# Autodesk Inventor assembly: mill_assembly
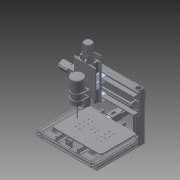
[picture p0: Inventor's stored thumbnail of the model, 180x180]
Saved by Autodesk Inventor 2014 (Build 180170000, 170)
## iProperties
Created: 2014-08-08
Part Number: mill_assembly
Document SubType Name: Assembly
Designer: Matthew
Author: Matthew
## Documents named in this file (29)
- C:\Users\Matthew\Documents\GitHub\CNC Mill\mill_assembly.iam
- C:\Users\Matthew\Documents\GitHub\CNC Mill\Imported Components\8020-2040\Assembly2.iam
- C:\Users\Matthew\Documents\GitHub\CNC Mill\8020\2020.ipt
- C:\Users\Matthew\Documents\GitHub\CNC Mill\8020\2020_18in.ipt
- C:\Users\Matthew\Documents\GitHub\CNC Mill\plate_4127.ipt
- C:\Users\Matthew\Documents\GitHub\CNC Mill\8020\gusset_4138.ipt
- C:\Users\Matthew\Documents\GitHub\CNC Mill\8020\gusset_4134.ipt
- C:\Users\Matthew\Documents\GitHub\CNC Mill\mic6_plate.ipt
- C:\Users\Matthew\Documents\GitHub\CNC Mill\1605\1605_400mm.ipt
- C:\Users\Matthew\Documents\GitHub\CNC Mill\1605\1605_ballnut.ipt
- C:\Users\Matthew\Documents\GitHub\CNC Mill\nema23_motor_mount.ipt
- C:\Users\Matthew\Documents\GitHub\CNC Mill\fk12.ipt
- C:\Users\Matthew\Documents\GitHub\CNC Mill\sbr\sbr20\SBR20UU.iam
- C:\Users\Matthew\Documents\GitHub\CNC Mill\6.35x10mm_coupler.ipt
- C:\Users\Matthew\Documents\GitHub\CNC Mill\sbr\sbr20\sbr20_400mm.ipt
- C:\Users\Matthew\Documents\GitHub\CNC Mill\HD16.ipt
- C:\Users\Matthew\Documents\GitHub\CNC Mill\nema23_HS8630.ipt
- C:\Users\Matthew\Documents\GitHub\CNC Mill\z-axis_mount_plate.ipt
- C:\Users\Matthew\Documents\GitHub\CNC Mill\1605\1605_200mm.ipt
- C:\Users\Matthew\Documents\GitHub\CNC Mill\y-axis_mount_plate.ipt
- C:\Users\Matthew\Documents\GitHub\CNC Mill\8020\2020_16in.ipt
- C:\Users\Matthew\Documents\GitHub\CNC Mill\router_plate.ipt
- C:\Users\Matthew\Documents\GitHub\CNC Mill\router_mount.ipt
- C:\Users\Matthew\Documents\GitHub\CNC Mill\1617evs.ipt
- C:\Users\Matthew\Documents\GitHub\CNC Mill\ff12_mount.ipt
- C:\Users\Matthew\Documents\GitHub\CNC Mill\ff12.ipt
- C:\Users\Matthew\Documents\GitHub\CNC Mill\sbr\sbr20\sbr20_500mm.ipt
- C:\Users\Matthew\Documents\GitHub\CNC Mill\1605\1605_500mm.ipt
- C:\Users\Matthew\Documents\GitHub\CNC Mill\sbr\sbr20\sbr20_300mm.ipt
## Components (69 placed, 28 different names)
1. Assembly2:1 [sub-assembly] — Mate:22, Mate:24, Mate:26, Mate:39, Mate:41, Mate:42, Mate:43, Mate:45, Mate:161, Flush:91, Flush:114, Flush:115, Mate:184, Flush:117, Flush:118
2. 2020_18in:1 — Mate:31, Mate:32, Mate:38, Mate:47, Mate:48, Mate:181, Flush:107, Flush:113, Flush:127, Mate:192, Flush:128
3. 2020_18in:2 — Mate:28, Mate:29, Mate:34, Mate:50, Mate:51, Mate:189, Flush:124, Flush:125
4. plate_4127:1 — Mate:39, Mate:41, Flush:119
5. gusset_4138:1 — Mate:22
6. gusset_4134:1 — Mate:28, Mate:29
7. gusset_4138:2 — Mate:24, Mate:26, Mate:207
8. gusset_4134:2 — Mate:31, Mate:32
9. gusset_4134:3 — Mate:34, Flush:61, Mate:193
10. gusset_4134:4 — Mate:38, Flush:62, Mate:191
11. plate_4127:2 — Mate:42, Mate:43, Mate:45, Flush:116
12. gusset_4134:5 — Mate:50, Mate:51
13. gusset_4134:6 — Mate:47, Mate:48, Flush:61, Flush:62
14. mic6_plate:1 — Flush:76, Flush:77, Mate:141
15. 1605_400mm:1 — Mate:98, Mate:100, Mate:108, Insert:2, Insert:13
16. 1605_ballnut:1 — Mate:108, Mate:133, Mate:134, Flush:75
17. nema23_motor_mount:1 — Mate:99, Mate:136, Mate:137, Mate:196, Flush:132
18. nema23_motor_mount:2 — Mate:153, Flush:86, Mate:154, Mate:155, Mate:156, Mate:157
19. 1605_ballnut:6 — Mate:150, Mate:158, Flush:90, Mate:159
20. fk12:1 — Mate:98, Mate:99, Mate:100, Mate:137
21. fk12:3 — Mate:156, Mate:157, Mate:214
22. SBR20UU:1 [sub-assembly] — Mate:131, Flush:69, Flush:70, Flush:73, Mate:138, Mate:140, Flush:77, Mate:141
23. 6.35x10mm_coupler:1 — Insert:3, Insert:4
24. sbr20_400mm:1 — Mate:130, Mate:198, Flush:136
25. SBR20UU:2 [sub-assembly] — Mate:129, Mate:132, Flush:71, Flush:72, Mate:139
26. sbr20_400mm:2 — Mate:129, Mate:197, Flush:136
27. SBR20UU:3 [sub-assembly] — Mate:130, Mate:131, Flush:69, Flush:70, Flush:74, Flush:76
28. SBR20UU:4 [sub-assembly] — Mate:132, Flush:71, Flush:72, Flush:73, Flush:74
29. HD16:1 — Mate:133, Mate:134, Flush:75, Mate:138, Mate:139, Mate:140
30. nema23_HS8630:1 — Mate:135, Mate:136
31. 6.35x10mm_coupler:2 — Insert:2, Mate:135
32. SBR20UU:5 [sub-assembly] — Flush:78, Flush:79, Mate:144, Flush:84, Flush:85, Mate:160
33. SBR20UU:6 [sub-assembly] — Flush:78, Flush:79, Mate:144, Mate:213
34. SBR20UU:7 [sub-assembly] — Flush:84, Flush:85
35. SBR20UU:8 [sub-assembly] — Mate:212
36. z-axis_mount_plate:1 — Mate:153, Flush:86, Mate:167, Flush:102, Flush:103, Mate:208, Mate:209, Flush:139
37. 1605_200mm:1 — Mate:150, Insert:3
38. nema23_HS8630:2 — Mate:154, Mate:155, Insert:4
39. HD16:6 — Mate:158, Flush:90, Mate:159, Mate:160, Mate:186, Flush:120, Flush:121, Mate:210, Mate:211
40. y-axis_mount_plate:1 — Mate:161, Flush:91, Mate:177, Mate:199, Mate:200, Flush:135, Mate:206, Flush:137
41. SBR20UU:9 [sub-assembly] — Flush:95, Flush:96, Flush:99, Flush:101, Mate:167, Flush:103, Mate:201
42. SBR20UU:10 [sub-assembly] — Flush:95, Flush:96, Mate:166, Flush:97, Flush:98, Flush:102
43. SBR20UU:11 [sub-assembly] — Flush:99, Flush:100, Flush:101
44. SBR20UU:12 [sub-assembly] — Mate:166, Flush:97, Flush:98, Flush:100, Mate:180, Mate:202
45. nema23_motor_mount:4 — Mate:177, Flush:137
46. fk12:4 — Insert:8, Mate:204, Insert:10
47. 6.35x10mm_coupler:3
48. nema23_HS8630:3
49. 1605_400mm:2 — Mate:176, Insert:8
50. 1605_ballnut:7 — Mate:176
51. HD16:7 — Mate:180, Mate:203, Mate:205
52. 2020_16in:1 — Mate:181, Flush:107, Flush:113, Flush:114, Flush:115, Mate:184, Flush:116, Mate:194, Flush:129, Flush:130, Mate:207
53. 2020_16in:2 — Flush:117, Flush:118, Flush:119, Mate:195, Flush:131
54. router_plate:1 — Mate:186, Flush:120, Flush:121, Mate:187, Flush:122, Flush:123
55. router_mount:1 — Insert:7, Mate:187, Flush:122, Flush:123
56. 1617evs:1 — Insert:7
57. ff12_mount:1 — Insert:9
58. ff12:1 — Insert:9, Insert:13
59. sbr20_500mm:1 — Flush:133, Mate:200, Mate:201, Mate:203, Mate:204, Flush:135
60. 2020_16in:3 — Mate:189, Flush:124, Flush:125, Flush:127, Mate:191, Mate:192, Flush:128, Mate:193, Mate:197, Mate:198, Mate:215, Mate:216, Flush:141
61. 2020_16in:4 — Mate:194, Flush:129, Flush:130, Mate:195, Flush:131, Mate:196, Flush:132, Flush:140
62. sbr20_500mm:2 — Flush:133, Mate:199, Mate:202, Mate:205
63. 1605_500mm:1 — Insert:10, Insert:11
64. ff12:2 — Insert:11, Insert:12
65. ff12_mount:2 — Insert:12, Mate:206
66. sbr20_300mm:1 — Flush:138, Mate:208, Mate:210, Mate:213, Mate:214, Flush:139
67. sbr20_300mm:2 — Flush:138, Mate:209, Mate:211, Mate:212
68. 2020:1 — Mate:215, Flush:140
69. 2020:2 — Mate:216, Flush:141
## Relationships (158: Mate 89, Flush 58, Insert 11)
- Mate:22: Assembly2:1 ↔ gusset_4138:1
- Mate:24: Assembly2:1 ↔ gusset_4138:2
- Mate:26: Assembly2:1 ↔ gusset_4138:2
- Mate:28: 2020_18in:2 ↔ gusset_4134:1
- Mate:29: 2020_18in:2 ↔ gusset_4134:1
- Mate:31: 2020_18in:1 ↔ gusset_4134:2
- Mate:32: 2020_18in:1 ↔ gusset_4134:2
- Mate:34: 2020_18in:2 ↔ gusset_4134:3
- Mate:38: 2020_18in:1 ↔ gusset_4134:4
- Mate:39: Assembly2:1 ↔ plate_4127:1
- Mate:41: Assembly2:1 ↔ plate_4127:1
- Mate:42: Assembly2:1 ↔ plate_4127:2
- Mate:43: Assembly2:1 ↔ plate_4127:2
- Mate:45: Assembly2:1 ↔ plate_4127:2
- Mate:47: 2020_18in:1 ↔ gusset_4134:6
- Mate:48: 2020_18in:1 ↔ gusset_4134:6
- Mate:50: 2020_18in:2 ↔ gusset_4134:5
- Mate:51: 2020_18in:2 ↔ gusset_4134:5
- Mate:98: 1605_400mm:1 ↔ fk12:1
- Mate:99: nema23_motor_mount:1 ↔ fk12:1
- Mate:100: 1605_400mm:1 ↔ fk12:1
- Mate:108: 1605_400mm:1 ↔ 1605_ballnut:1
- Flush:61: gusset_4134:3 ↔ gusset_4134:6
- Flush:62: gusset_4134:4 ↔ gusset_4134:6
- Mate:129: SBR20UU:2 ↔ sbr20_400mm:2
- Mate:130: sbr20_400mm:1 ↔ SBR20UU:3
- Mate:131 (20 mm): SBR20UU:1 ↔ SBR20UU:3
- Flush:69: SBR20UU:1 ↔ SBR20UU:3
- Flush:70: SBR20UU:1 ↔ SBR20UU:3
- Mate:132 (20 mm): SBR20UU:2 ↔ SBR20UU:4
- Flush:71: SBR20UU:2 ↔ SBR20UU:4
- Flush:72: SBR20UU:2 ↔ SBR20UU:4
- Flush:73: SBR20UU:1 ↔ SBR20UU:4
- Flush:74: SBR20UU:3 ↔ SBR20UU:4
- Mate:133: 1605_ballnut:1 ↔ HD16:1
- Mate:134: 1605_ballnut:1 ↔ HD16:1
- Flush:75: 1605_ballnut:1 ↔ HD16:1
- Insert:2 (-12.5 mm): 1605_400mm:1 ↔ 6.35x10mm_coupler:2
- Mate:135: nema23_HS8630:1 ↔ 6.35x10mm_coupler:2
- Mate:136: nema23_motor_mount:1 ↔ nema23_HS8630:1
- Mate:137: nema23_motor_mount:1 ↔ fk12:1
- Mate:138 (42.3 mm): SBR20UU:1 ↔ HD16:1
- Mate:139 (42.3 mm): SBR20UU:2 ↔ HD16:1
- Mate:140 (-7.5 mm): SBR20UU:1 ↔ HD16:1
- Flush:76 (38.1 mm): mic6_plate:1 ↔ SBR20UU:3
- Flush:77 (-92.4052 mm): mic6_plate:1 ↔ SBR20UU:1
- Mate:141: mic6_plate:1 ↔ SBR20UU:1
- Flush:78: SBR20UU:5 ↔ SBR20UU:6
- Flush:79: SBR20UU:5 ↔ SBR20UU:6
- Mate:144 (10 mm): SBR20UU:5 ↔ SBR20UU:6
- [Flush]: SBR20UU:7 ↔ SBR20UU:8
- [Flush]: SBR20UU:7 ↔ SBR20UU:8
- [Mate] (10 mm): SBR20UU:7 ↔ SBR20UU:8
- Flush:84: SBR20UU:5 ↔ SBR20UU:7
- Flush:85: SBR20UU:5 ↔ SBR20UU:7
- Mate:150: 1605_ballnut:6 ↔ 1605_200mm:1
- Insert:3 (-12.5 mm): 6.35x10mm_coupler:1 ↔ 1605_200mm:1
- Mate:153: nema23_motor_mount:2 ↔ z-axis_mount_plate:1
- Flush:86: nema23_motor_mount:2 ↔ z-axis_mount_plate:1
- Mate:154: nema23_motor_mount:2 ↔ nema23_HS8630:2
- Mate:155: nema23_motor_mount:2 ↔ nema23_HS8630:2
- Insert:4 (-7 mm): 6.35x10mm_coupler:1 ↔ nema23_HS8630:2
- Mate:156: nema23_motor_mount:2 ↔ fk12:3
- Mate:157: nema23_motor_mount:2 ↔ fk12:3
- Mate:158: 1605_ballnut:6 ↔ HD16:6
- Flush:90: 1605_ballnut:6 ↔ HD16:6
- Mate:159: 1605_ballnut:6 ↔ HD16:6
- Mate:160 (-12.5 mm): SBR20UU:5 ↔ HD16:6
- Mate:161: Assembly2:1 ↔ y-axis_mount_plate:1
- Flush:91: Assembly2:1 ↔ y-axis_mount_plate:1
- Flush:95: SBR20UU:9 ↔ SBR20UU:10
- Flush:96: SBR20UU:9 ↔ SBR20UU:10
- Mate:166 (60 mm): SBR20UU:10 ↔ SBR20UU:12
- Flush:97: SBR20UU:10 ↔ SBR20UU:12
- Flush:98: SBR20UU:10 ↔ SBR20UU:12
- Flush:99: SBR20UU:9 ↔ SBR20UU:11
- Flush:100: SBR20UU:11 ↔ SBR20UU:12
- Flush:101: SBR20UU:9 ↔ SBR20UU:11
- Mate:167: z-axis_mount_plate:1 ↔ SBR20UU:9
- Flush:102: z-axis_mount_plate:1 ↔ SBR20UU:10
- Flush:103: z-axis_mount_plate:1 ↔ SBR20UU:9
- [Mate]: nema23_motor_mount:4 ↔ nema23_HS8630:3
- [Mate]: nema23_motor_mount:4 ↔ nema23_HS8630:3
- [Insert] (-7 mm): 6.35x10mm_coupler:3 ↔ nema23_HS8630:3
- [Mate]: nema23_motor_mount:4 ↔ fk12:4
- [Mate]: nema23_motor_mount:4 ↔ fk12:4
- [Mate]: 1605_ballnut:7 ↔ HD16:7
- [Flush]: 1605_ballnut:7 ↔ HD16:7
- [Mate]: 1605_ballnut:7 ↔ HD16:7
- Mate:176: 1605_400mm:2 ↔ 1605_ballnut:7
- Mate:177: y-axis_mount_plate:1 ↔ nema23_motor_mount:4
- Mate:180 (12.5 mm): SBR20UU:12 ↔ HD16:7
- Mate:181: 2020_18in:1 ↔ 2020_16in:1
- Flush:107: 2020_18in:1 ↔ 2020_16in:1
- Flush:113: 2020_18in:1 ↔ 2020_16in:1
- Flush:114: Assembly2:1 ↔ 2020_16in:1
- Flush:115: Assembly2:1 ↔ 2020_16in:1
- Mate:184: Assembly2:1 ↔ 2020_16in:1
- Flush:116: plate_4127:2 ↔ 2020_16in:1
- Flush:117: Assembly2:1 ↔ 2020_16in:2
- Flush:118: Assembly2:1 ↔ 2020_16in:2
- Flush:119: plate_4127:1 ↔ 2020_16in:2
- Insert:7: router_mount:1 ↔ 1617evs:1
- Mate:186: HD16:6 ↔ router_plate:1
- Flush:120 (-96.7994 mm): HD16:6 ↔ router_plate:1
- Flush:121 (64.897 mm): HD16:6 ↔ router_plate:1
- Mate:187: router_plate:1 ↔ router_mount:1
- Flush:122: router_plate:1 ↔ router_mount:1
- Flush:123 (44.45 mm): router_plate:1 ↔ router_mount:1
- Insert:8: fk12:4 ↔ 1605_400mm:2
- Insert:9: ff12_mount:1 ↔ ff12:1
- Mate:189: 2020_18in:2 ↔ 2020_16in:3
- Flush:124: 2020_18in:2 ↔ 2020_16in:3
- Flush:125: 2020_18in:2 ↔ 2020_16in:3
- Flush:127: 2020_18in:1 ↔ 2020_16in:3
- Mate:191: gusset_4134:4 ↔ 2020_16in:3
- Mate:192: 2020_18in:1 ↔ 2020_16in:3
- Flush:128: 2020_18in:1 ↔ 2020_16in:3
- Mate:193: gusset_4134:3 ↔ 2020_16in:3
- Mate:194: 2020_16in:1 ↔ 2020_16in:4
- Flush:129: 2020_16in:1 ↔ 2020_16in:4
- Flush:130: 2020_16in:1 ↔ 2020_16in:4
- Mate:195: 2020_16in:2 ↔ 2020_16in:4
- Flush:131: 2020_16in:2 ↔ 2020_16in:4
- Mate:196: nema23_motor_mount:1 ↔ 2020_16in:4
- Flush:132: nema23_motor_mount:1 ↔ 2020_16in:4
- Mate:197: sbr20_400mm:2 ↔ 2020_16in:3
- Mate:198: sbr20_400mm:1 ↔ 2020_16in:3
- Flush:133: sbr20_500mm:1 ↔ sbr20_500mm:2
- Mate:199: y-axis_mount_plate:1 ↔ sbr20_500mm:2
- Mate:200: y-axis_mount_plate:1 ↔ sbr20_500mm:1
- Mate:201: SBR20UU:9 ↔ sbr20_500mm:1
- Mate:202: SBR20UU:12 ↔ sbr20_500mm:2
- Mate:203 (19.9 mm): HD16:7 ↔ sbr20_500mm:1
- Mate:204 (-40 mm): fk12:4 ↔ sbr20_500mm:1
- Mate:205 (19.9 mm): HD16:7 ↔ sbr20_500mm:2
- Flush:135: y-axis_mount_plate:1 ↔ sbr20_500mm:1
- Flush:136: sbr20_400mm:1 ↔ sbr20_400mm:2
- Insert:10: fk12:4 ↔ 1605_500mm:1
- Insert:11: 1605_500mm:1 ↔ ff12:2
- Insert:12: ff12:2 ↔ ff12_mount:2
- Mate:206: y-axis_mount_plate:1 ↔ ff12_mount:2
- Insert:13: 1605_400mm:1 ↔ ff12:1
- Flush:137: y-axis_mount_plate:1 ↔ nema23_motor_mount:4
- Mate:207: gusset_4138:2 ↔ 2020_16in:1
- Flush:138: sbr20_300mm:1 ↔ sbr20_300mm:2
- Mate:208: z-axis_mount_plate:1 ↔ sbr20_300mm:1
- Mate:209: z-axis_mount_plate:1 ↔ sbr20_300mm:2
- Mate:210 (11 mm): HD16:6 ↔ sbr20_300mm:1
- Mate:211 (11 mm): HD16:6 ↔ sbr20_300mm:2
- Mate:212: SBR20UU:8 ↔ sbr20_300mm:2
- Mate:213: SBR20UU:6 ↔ sbr20_300mm:1
- Mate:214 (-40 mm): fk12:3 ↔ sbr20_300mm:1
- Flush:139: z-axis_mount_plate:1 ↔ sbr20_300mm:1
- Mate:215: 2020_16in:3 ↔ 2020:1
- Flush:140: 2020_16in:4 ↔ 2020:1
- Mate:216: 2020_16in:3 ↔ 2020:2
- Flush:141: 2020_16in:3 ↔ 2020:2
## Named parameters: mountspace = 20 mm, yoffset = 42.3 mm, d321_d318 = 0 mm, d322_d319 = 0 mm, d323_d320 = 10 mm, yaxisspacing = 60 mm, d373_d340 = -7 mm, d374_d341 = 0 mm, d375_d342 = 0 mm, d376_d338 = 0 mm, d377_d339 = 0 mm, d379_d346 = 0 mm, d380_d347 = 0 mm, d381_d348 = 0 mm, yaxissbrspacing = 19.9 mm
